# Autodesk Inventor assembly: Assembly_Cube_v4_polfilter
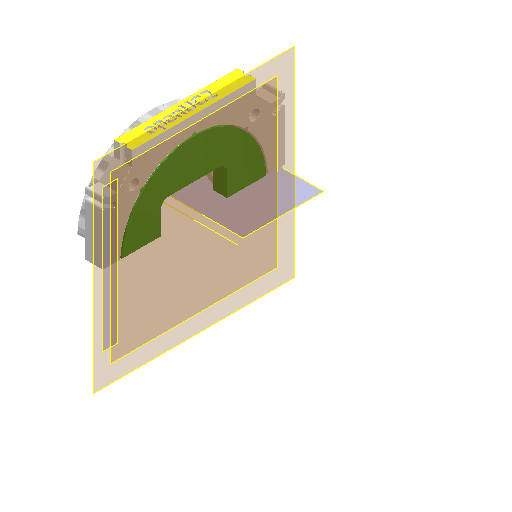
[picture p0: Inventor's stored thumbnail of the model, 512x512]
Saved by Autodesk Inventor 2025.1 (Build 291241000, 241)
## iProperties
Created: 2024-10-03
Part Number: Assembly_Cube_v4_polfilter
Document SubType Name: Assembly
Designer: diederichbenedict
Author: diederichbenedict
## Documents named in this file (6)
- C:\Users\Muriel\Documents\GitHub\TechnicalDocs-openUC2-QBox\Production_Files\CAD_Files\INVENTOR\Assembly_Cube_v4_polfilter.iam
- C:\Users\Muriel\Documents\GitHub\TechnicalDocs-openUC2-QBox\Production_Files\CAD_Files\INVENTOR\Assembly_Cube_v4.iam
- C:\Users\Muriel\Documents\GitHub\TechnicalDocs-openUC2-QBox\Production_Files\CAD_Files\INVENTOR\10_Insert_v4.ipt
- C:\Users\Muriel\Documents\GitHub\TechnicalDocs-openUC2-QBox\Production_Files\CAD_Files\INVENTOR\20_Cube_4_insert_polfilter_base.ipt
- C:\Users\Muriel\Documents\GitHub\TechnicalDocs-openUC2-QBox\Production_Files\CAD_Files\INVENTOR\00_Polfilter_rectangular_20mm.ipt
- C:\Users\Muriel\Documents\GitHub\TechnicalDocs-openUC2-QBox\Production_Files\CAD_Files\INVENTOR\20_Cube_4_insert_polfilter_nut.ipt
## Components (5 placed, 5 different names)
1. Assembly_Cube_v4:1 [sub-assembly] — Mate:1, Mate:2
2. 10_Insert_v4:2
3. 20_Cube_4_insert_polfilter_base:1 — Flush:6, Mate:9, Flush:7, Mate:10
4. 00_Polfilter_rectangular_20mm:1
5. 20_Cube_4_insert_polfilter_nut:1 — Flush:6, Mate:9, Flush:7, Mate:10
## Relationships (8: Mate 4, Flush 3, Angle 1)
- Mate:1: Assembly_Cube_v4:1
- Mate:2: Assembly_Cube_v4:1
- [Flush]: 10_Insert_v4:2 ↔ 20_Cube_4_insert_polfilter_base:1
- [Angle] (180 deg): 10_Insert_v4:2 ↔ 20_Cube_4_insert_polfilter_base:1
- Flush:6: 20_Cube_4_insert_polfilter_base:1 ↔ 20_Cube_4_insert_polfilter_nut:1
- Mate:9: 20_Cube_4_insert_polfilter_base:1 ↔ 20_Cube_4_insert_polfilter_nut:1
- Flush:7: 20_Cube_4_insert_polfilter_base:1 ↔ 20_Cube_4_insert_polfilter_nut:1
- Mate:10: 20_Cube_4_insert_polfilter_base:1 ↔ 20_Cube_4_insert_polfilter_nut:1
## Named parameters: d18_d10 = 0 mm, d19_d15 = 180 deg
